# Autodesk Inventor assembly: Assy_cover_front
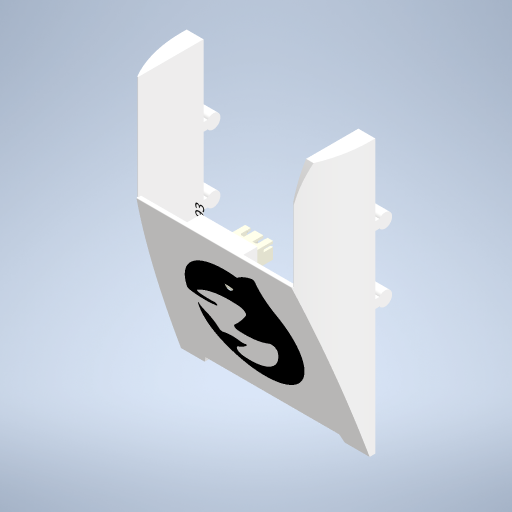
[picture p0: Inventor's stored thumbnail of the model, 512x512]
Saved by Autodesk Inventor 2024.1 (Build 281209000, 209)
## iProperties
Created: 2025-03-07
Part Number: Assy_cover_front
Document SubType Name: Assembly
Designer: hibik
Author: hibik
## Documents named in this file (4)
- C:\Users\hibik\Documents\Robomech\RESCUE\ORCA\hard\cover\Assy_cover_front.iam
- C:\Users\hibik\Documents\Robomech\RESCUE\ORCA\hard\cover\cover_front.ipt
- C:\Users\hibik\Documents\Robomech\RESCUE\ORCA\hard\cover\ROGO_front_cover.ipt
- C:\Users\hibik\Documents\Robomech\RESCUE\ORCA\hard\board\CORE_model\external_io_led.iam
## Components (3 placed, 3 different names)
1. cover_front:1 — フラッシュ:3, 挿入:1, 角度:1
2. ROGO_front_cover:1 — フラッシュ:2, フラッシュ:3
3. external_io_led:1 [sub-assembly] — 挿入:1, 角度:1
## Relationships (4: Flush 2, Insert 1, Angle 1)
- フラッシュ:2 [Flush]: ROGO_front_cover:1
- フラッシュ:3 [Flush] (30 mm): cover_front:1 ↔ ROGO_front_cover:1
- 挿入:1 [Insert]: cover_front:1 ↔ external_io_led:1
- 角度:1 [Angle] (0 deg): cover_front:1 ↔ external_io_led:1
